# Autodesk Inventor assembly: holder_assembly
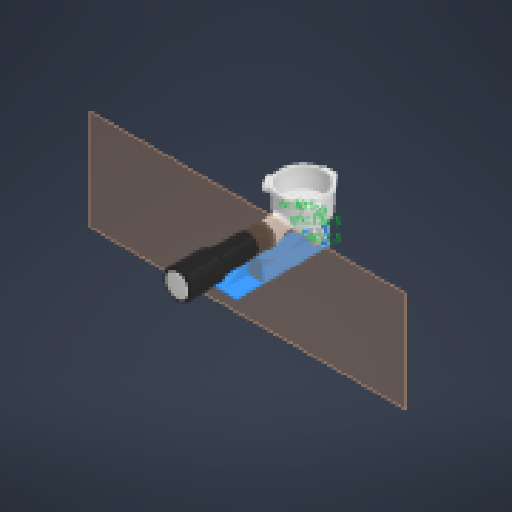
[picture p0: Inventor's stored thumbnail of the model, 512x512]
Saved by Autodesk Inventor 2026 (Build 300175000, 175)
## iProperties
Created: 2025-04-17
Part Number: holder_assembly
Document SubType Name: Assembly
Designer: Paul Juschitz
Author: Paul Juschitz
## Documents named in this file (3)
- C:\Users\Paul Juschitz\Documents\private\m5_GBW_mod\M5_GBW_mod\CAD\holder_assembly.iam
- C:\Users\Paul Juschitz\Documents\private\m5_GBW_mod\M5_GBW_mod\CAD\downloads\portafilter\BES870XL Portafilter\BES870XL Portafilter\BES870XL Portafilter_assembled.iam
- C:\Users\Paul Juschitz\Documents\private\m5_GBW_mod\M5_GBW_mod\CAD\my_portafilter_holder_4.ipt
## Components (2 placed, 2 different names)
1. BES870XL Portafilter_assembled:1 [sub-assembly] — Angle:1, Angle:2, Mate:1, Tangent:1
2. my_portafilter_holder_4:1 — Angle:1, Angle:2, Mate:1, Tangent:1, Flush:1
## Relationships (5: Angle 2, Mate 1, Tangent 1, Flush 1)
- Angle:1 (180 deg): BES870XL Portafilter_assembled:1 ↔ my_portafilter_holder_4:1
- Angle:2 (180 deg): BES870XL Portafilter_assembled:1 ↔ my_portafilter_holder_4:1
- Mate:1: BES870XL Portafilter_assembled:1 ↔ my_portafilter_holder_4:1
- Tangent:1: BES870XL Portafilter_assembled:1 ↔ my_portafilter_holder_4:1
- Flush:1: my_portafilter_holder_4:1
